# Autodesk Inventor assembly: Assembly_Lambda_2_rotator
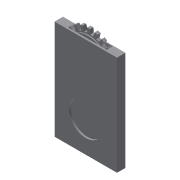
[picture p0: Inventor's stored thumbnail of the model, 180x180]
Saved by Autodesk Inventor 2019 (Build 230136000, 136)
## iProperties
Created: 2019-07-08
Part Number: Assembly_Lambda_2_rotator
Document SubType Name: Assembly
Designer: diederichbenedict
Author: diederichbenedict
## Documents named in this file (6)
- C:\Users\diederichbenedict\Dropbox\Dokumente\Promotion\PROJECTS\STORMoChip\INVENTOR\Nanoscopy-on-a-cheap\Assembly_Lambda_2_rotator.iam
- C:\Users\diederichbenedict\Dropbox\Dokumente\Promotion\PROJECTS\STORMoChip\INVENTOR\Nanoscopy-on-a-cheap\00_Lambda_2_Plate.ipt
- C:\Users\diederichbenedict\Dropbox\Dokumente\Promotion\PROJECTS\STORMoChip\INVENTOR\Nanoscopy-on-a-cheap\200_Holder_Lambdaplate_1.ipt
- C:\Users\diederichbenedict\Dropbox\Dokumente\Promotion\PROJECTS\STORMoChip\INVENTOR\Nanoscopy-on-a-cheap\200_Gearbox.ipt
- C:\Users\diederichbenedict\Dropbox\Dokumente\Promotion\PROJECTS\STORMoChip\INVENTOR\Nanoscopy-on-a-cheap\200_Lambdaplatte_2_conterplate.ipt
- C:\Users\diederichbenedict\Dropbox\Dokumente\Promotion\PROJECTS\STORMoChip\INVENTOR\Nanoscopy-on-a-cheap\200_Gearbox_conterplate.ipt
## Components (7 placed, 5 different names)
1. 00_Lambda_2_Plate:1 — Flush:1
2. 200_Holder_Lambdaplate_1:1 — Flush:1, Flush:3, Flush:4
3. 200_Holder_Lambdaplate_1:2 — Mate:1, Insert:1
4. 200_Gearbox:1 — Flush:3, Flush:5, Flush:6
5. 200_Lambdaplatte_2_conterplate:1 — Flush:4
6. 200_Gearbox_conterplate:1 — Flush:5, Flush:6
7. 200_Lambdaplatte_2_conterplate:2 — Mate:1, Insert:1
## Relationships (7: Flush 5, Mate 1, Insert 1)
- Flush:1: 00_Lambda_2_Plate:1 ↔ 200_Holder_Lambdaplate_1:1
- Flush:3: 200_Holder_Lambdaplate_1:1 ↔ 200_Gearbox:1
- Flush:4: 200_Holder_Lambdaplate_1:1 ↔ 200_Lambdaplatte_2_conterplate:1
- Flush:5: 200_Gearbox:1 ↔ 200_Gearbox_conterplate:1
- Flush:6: 200_Gearbox:1 ↔ 200_Gearbox_conterplate:1
- Mate:1: 200_Holder_Lambdaplate_1:2 ↔ 200_Lambdaplatte_2_conterplate:2
- Insert:1: 200_Holder_Lambdaplate_1:2 ↔ 200_Lambdaplatte_2_conterplate:2
